# Autodesk Inventor assembly: アーム3
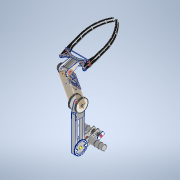
[picture p0: Inventor's stored thumbnail of the model, 180x180]
Saved by Autodesk Inventor 2021 (Build 250183000, 183)
## iProperties
Created: 2022-02-03
Part Number: アーム3
Document SubType Name: Assembly
Designer: hirohumi
Mass: 1757.85 g
Surface Area: 6806.39 cm^2
Volume: 1186.66 cm^3
Density: 1.48134 g/cm^3
Author: hirohumi
## Documents named in this file (25)
- C:\Users\hirohumi\OneDrive\ドキュメント\ロボ研\2022NHKロボコン\R2_version1\3軸アームver3\アーム3.iam
- C:\Users\hirohumi\OneDrive\ドキュメント\ロボ研\2022NHKロボコン\R2_version1\3軸アームver3\アーム3_角柱1.ipt
- C:\Users\hirohumi\OneDrive\ドキュメント\ロボ研\2022NHKロボコン\R2_version1\3軸アームver3\関節3_側板右.ipt
- C:\Users\hirohumi\OneDrive\ドキュメント\ロボ研\2022NHKロボコン\R2_version1\3軸アームver3\関節3_側板左.ipt
- C:\Users\hirohumi\OneDrive\ドキュメント\ロボ研\2022NHKロボコン\R2_version1\RS-555-71.ipt
- C:\Users\hirohumi\OneDrive\ドキュメント\ロボ研\2022NHKロボコン\R2_version1\3軸アーム\カップリング_軸6mm.ipt
- C:\Users\hirohumi\OneDrive\ドキュメント\ロボ研\2022NHKロボコン\R2_version1\3軸アーム\カップリング_軸8mm_2.5mm.ipt
- C:\Users\hirohumi\OneDrive\ドキュメント\ロボ研\2022NHKロボコン\R2_version1\3軸アーム\軸8-30.ipt
- C:\Users\hirohumi\OneDrive\ドキュメント\ロボ研\2022NHKロボコン\R2_version1\3軸アーム\プーリ_歯数15.ipt
- C:\Users\hirohumi\OneDrive\ドキュメント\ロボ研\2022NHKロボコン\R2_version1\3軸アーム\プーリ_歯数15_2.5mm.ipt
- C:\Users\hirohumi\OneDrive\ドキュメント\ロボ研\2022NHKロボコン\R2_version1\3軸アーム\カップリング_軸8mm.ipt
- C:\Users\hirohumi\OneDrive\ドキュメント\ロボ研\2022NHKロボコン\R2_version1\3軸アーム\AMT102Normal\CUI_DEVICES_AMT102-0048-N8000-S.iam
- C:\Users\hirohumi\OneDrive\ドキュメント\ロボ研\2022NHKロボコン\R2_version1\3軸アーム\エンコーダマウント.ipt
- C:\Users\hirohumi\OneDrive\ドキュメント\ロボ研\2022NHKロボコン\R2_version1\3軸アームver2\関節3_プーリ側板.ipt
- C:\Users\hirohumi\OneDrive\ドキュメント\ロボ研\2022NHKロボコン\R2_version1\3軸アーム\ベアリングフランジ付き.ipt
- C:\Users\hirohumi\OneDrive\ドキュメント\ロボ研\2022NHKロボコン\R2_version1\3軸アーム\ギア_歯数50.ipt
- C:\Users\hirohumi\OneDrive\ドキュメント\ロボ研\2022NHKロボコン\R2_version1\RS-775GM104 v1.ipt
- C:\Users\hirohumi\OneDrive\ドキュメント\ロボ研\2022NHKロボコン\R2_version1\3軸アームver3\関節3_前側板.ipt
- C:\Users\hirohumi\OneDrive\ドキュメント\ロボ研\2022NHKロボコン\R2_version1\3軸アーム\プーリ_歯数60.ipt
- C:\Users\hirohumi\OneDrive\ドキュメント\ロボ研\2022NHKロボコン\R2_version1\3軸アーム\関節1_プーリ2個.iam
- C:\Users\hirohumi\OneDrive\ドキュメント\ロボ研\2022NHKロボコン\R2_version1\3軸アーム\軸8-80.ipt
- C:\Users\hirohumi\OneDrive\ドキュメント\ロボ研\2022NHKロボコン\R2_version1\3軸アームver2\関節2_側板.ipt
- C:\Users\hirohumi\OneDrive\ドキュメント\ロボ研\2022NHKロボコン\R2_version1\3軸アームver2\関節2_上板.ipt
- C:\Users\hirohumi\OneDrive\ドキュメント\ロボ研\2022NHKロボコン\R2_version1\R2_ハンド.iam
- C:\Users\hirohumi\OneDrive\ドキュメント\ロボ研\2022NHKロボコン\R2_version1\3軸アームver3\軸_6-30.ipt
## Components (50 placed, 24 different names)
1. アーム3_角柱1:1 — 挿入:62, 挿入:63, 挿入:64, 挿入:65, 挿入:81, 挿入:83, 挿入:85
2. アーム3_角柱1:2 — 挿入:82, 挿入:84, 挿入:86
3. 関節3_側板右:1 — 挿入:83, 挿入:84, 挿入:85, 挿入:86, 挿入:87, 挿入:88, 挿入:89, 挿入:90, 挿入:105, 挿入:106, 挿入:109, 挿入:110
4. 関節3_側板左:1 — 挿入:81, 挿入:82, 挿入:95, 挿入:96, 挿入:97, 挿入:98, 挿入:99, 挿入:100
5. RS-555-71:1 — 挿入:100
6. カップリング_軸6mm:1
7. カップリング_軸8mm_2.5mm:1
8. 軸8-30:1
9. プーリ_歯数15:1
10. プーリ_歯数15_2.5mm:1
11. カップリング_軸8mm:1 — 挿入:108
12. CUI_DEVICES_AMT102-0048-N8000-S:1 [sub-assembly]
13. エンコーダマウント:1 — 挿入:98, 挿入:99
14. 関節3_プーリ側板:1 — 挿入:91, 挿入:92, 挿入:93, 挿入:94
15. ベアリングフランジ付き:1 — 挿入:107
16. ギア_歯数50:1 — 挿入:109, 挿入:110
17. RS-775GM104 v1:1 — 挿入:89, 挿入:90
18. カップリング_軸8mm:2
19. カップリング_軸8mm_2.5mm:2
20. プーリ_歯数15:2
21. プーリ_歯数15_2.5mm:2 — 挿入:107
22. カップリング_軸8mm:3
23. CUI_DEVICES_AMT102-0048-N8000-S:2 [sub-assembly]
24. エンコーダマウント:2 — 挿入:87, 挿入:88
25. ベアリングフランジ付き:2 — 挿入:97
26. 関節3_プーリ側板:2 — 挿入:101, 挿入:102, 挿入:103, 挿入:104
27. ベアリングフランジ付き:3 — 挿入:108
28. 関節3_前側板:1 — 挿入:64, 挿入:65, 挿入:67
29. 関節3_前側板:2 — 挿入:62, 挿入:63, 挿入:66
30. ベアリングフランジ付き:4 — 挿入:66, メイト:3, メイト:6
31. ベアリングフランジ付き:5 — 挿入:67
32. プーリ_歯数60:1 — メイト:6
33. プーリ_歯数60:2 — 挿入:76, 挿入:77
34. 関節1_プーリ2個:1 [sub-assembly] — 挿入:78
35. 軸8-80:1
36. 軸8-80:2
37. 関節2_側板:1 — 挿入:74, 挿入:75, 挿入:76, 挿入:77, 挿入:79, メイト:5
38. 関節2_側板:2 — 挿入:80
39. 軸8-80:3 — 挿入:75, メイト:4
40. 軸8-80:4 — 挿入:74, メイト:3, 挿入:78
41. 関節2_上板:1 — 挿入:79, 挿入:80
42. R2_ハンド:1 [sub-assembly] — メイト:4, メイト:5
43. 軸_6-30:1 — 挿入:91, 挿入:95
44. 軸_6-30:2 — 挿入:92
45. 軸_6-30:3 — 挿入:93, 挿入:96
46. 軸_6-30:4 — 挿入:94
47. 軸_6-30:5 — 挿入:104
48. 軸_6-30:6 — 挿入:103
49. 軸_6-30:7 — 挿入:102, 挿入:106
50. 軸_6-30:8 — 挿入:101, 挿入:105
## Relationships (74: Insert 70, Mate 4)
- [Insert]: カップリング_軸6mm:1 ↔ カップリング_軸8mm_2.5mm:1
- [Insert]: カップリング_軸6mm:1 ↔ カップリング_軸8mm_2.5mm:1
- [Insert]: RS-555-71:1 ↔ カップリング_軸6mm:1
- [Insert]: カップリング_軸6mm:1 ↔ 軸8-30:1
- [Insert]: プーリ_歯数15:1 ↔ プーリ_歯数15_2.5mm:1
- [Insert]: プーリ_歯数15:1 ↔ プーリ_歯数15_2.5mm:1
- [Insert]: プーリ_歯数15:1 ↔ カップリング_軸8mm:1
- [Insert]: プーリ_歯数15:1 ↔ カップリング_軸8mm:1
- [Insert]: CUI_DEVICES_AMT102-0048-N8000-S:1 ↔ エンコーダマウント:1
- [Insert]: CUI_DEVICES_AMT102-0048-N8000-S:1 ↔ エンコーダマウント:1
- [Insert]: 関節3_プーリ側板:1 ↔ ベアリングフランジ付き:1
- [Insert]: カップリング_軸8mm:2 ↔ カップリング_軸8mm_2.5mm:2
- [Insert]: カップリング_軸8mm:2 ↔ カップリング_軸8mm_2.5mm:2
- [Insert]: RS-775GM104 v1:1 ↔ カップリング_軸8mm_2.5mm:2
- [Insert]: プーリ_歯数15:2 ↔ プーリ_歯数15_2.5mm:2
- [Insert]: プーリ_歯数15:2 ↔ プーリ_歯数15_2.5mm:2
- [Insert]: プーリ_歯数15:2 ↔ カップリング_軸8mm:3
- [Insert]: プーリ_歯数15:2 ↔ カップリング_軸8mm:3
- [Insert]: CUI_DEVICES_AMT102-0048-N8000-S:2 ↔ エンコーダマウント:2
- [Insert]: CUI_DEVICES_AMT102-0048-N8000-S:2 ↔ エンコーダマウント:2
- [Insert]: 関節3_プーリ側板:2 ↔ ベアリングフランジ付き:3
- 挿入:62 [Insert]: アーム3_角柱1:1 ↔ 関節3_前側板:2
- 挿入:63 [Insert]: アーム3_角柱1:1 ↔ 関節3_前側板:2
- 挿入:64 [Insert]: アーム3_角柱1:1 ↔ 関節3_前側板:1
- 挿入:65 [Insert]: アーム3_角柱1:1 ↔ 関節3_前側板:1
- 挿入:66 [Insert]: 関節3_前側板:2 ↔ ベアリングフランジ付き:4
- 挿入:67 [Insert]: 関節3_前側板:1 ↔ ベアリングフランジ付き:5
- [Insert]: プーリ_歯数60:1 ↔ プーリ_歯数60:2
- [Insert]: プーリ_歯数60:1 ↔ プーリ_歯数60:2
- [Insert]: 軸8-80:1 ↔ 関節2_側板:1
- [Insert]: 軸8-80:2 ↔ 関節2_側板:1
- [Insert]: 軸8-80:1 ↔ 関節2_側板:2
- [Insert]: 軸8-80:2 ↔ 関節2_側板:2
- 挿入:74 [Insert]: 関節2_側板:1 ↔ 軸8-80:4
- 挿入:75 [Insert]: 関節2_側板:1 ↔ 軸8-80:3
- メイト:3 [Mate]: ベアリングフランジ付き:4 ↔ 軸8-80:4
- 挿入:76 [Insert]: プーリ_歯数60:2 ↔ 関節2_側板:1
- 挿入:77 [Insert]: プーリ_歯数60:2 ↔ 関節2_側板:1
- 挿入:78 [Insert]: 関節1_プーリ2個:1 ↔ 軸8-80:4
- 挿入:79 [Insert]: 関節2_側板:1 ↔ 関節2_上板:1
- 挿入:80 [Insert]: 関節2_側板:2 ↔ 関節2_上板:1
- メイト:4 [Mate]: 軸8-80:3 ↔ R2_ハンド:1
- メイト:5 [Mate]: 関節2_側板:1 ↔ R2_ハンド:1
- メイト:6 [Mate]: ベアリングフランジ付き:4 ↔ プーリ_歯数60:1
- 挿入:81 [Insert]: アーム3_角柱1:1 ↔ 関節3_側板左:1
- 挿入:82 [Insert]: アーム3_角柱1:2 ↔ 関節3_側板左:1
- 挿入:83 [Insert]: アーム3_角柱1:1 ↔ 関節3_側板右:1
- 挿入:84 [Insert]: アーム3_角柱1:2 ↔ 関節3_側板右:1
- 挿入:85 [Insert]: アーム3_角柱1:1 ↔ 関節3_側板右:1
- 挿入:86 [Insert]: アーム3_角柱1:2 ↔ 関節3_側板右:1
- 挿入:87 [Insert]: 関節3_側板右:1 ↔ エンコーダマウント:2
- 挿入:88 [Insert]: 関節3_側板右:1 ↔ エンコーダマウント:2
- 挿入:89 [Insert]: 関節3_側板右:1 ↔ RS-775GM104 v1:1
- 挿入:90 [Insert]: 関節3_側板右:1 ↔ RS-775GM104 v1:1
- 挿入:91 [Insert]: 関節3_プーリ側板:1 ↔ 軸_6-30:1
- 挿入:92 [Insert]: 関節3_プーリ側板:1 ↔ 軸_6-30:2
- 挿入:93 [Insert]: 関節3_プーリ側板:1 ↔ 軸_6-30:3
- 挿入:94 [Insert]: 関節3_プーリ側板:1 ↔ 軸_6-30:4
- 挿入:95 [Insert]: 関節3_側板左:1 ↔ 軸_6-30:1
- 挿入:96 [Insert]: 関節3_側板左:1 ↔ 軸_6-30:3
- 挿入:97 [Insert]: 関節3_側板左:1 ↔ ベアリングフランジ付き:2
- 挿入:98 [Insert]: 関節3_側板左:1 ↔ エンコーダマウント:1
- 挿入:99 [Insert]: 関節3_側板左:1 ↔ エンコーダマウント:1
- 挿入:100 [Insert]: 関節3_側板左:1 ↔ RS-555-71:1
- 挿入:101 [Insert]: 関節3_プーリ側板:2 ↔ 軸_6-30:8
- 挿入:102 [Insert]: 関節3_プーリ側板:2 ↔ 軸_6-30:7
- 挿入:103 [Insert]: 関節3_プーリ側板:2 ↔ 軸_6-30:6
- 挿入:104 [Insert]: 関節3_プーリ側板:2 ↔ 軸_6-30:5
- 挿入:105 [Insert]: 関節3_側板右:1 ↔ 軸_6-30:8
- 挿入:106 [Insert]: 関節3_側板右:1 ↔ 軸_6-30:7
- 挿入:107 [Insert]: ベアリングフランジ付き:1 ↔ プーリ_歯数15_2.5mm:2
- 挿入:108 [Insert]: カップリング_軸8mm:1 ↔ ベアリングフランジ付き:3
- 挿入:109 [Insert]: 関節3_側板右:1 ↔ ギア_歯数50:1
- 挿入:110 [Insert]: 関節3_側板右:1 ↔ ギア_歯数50:1
## Named parameters: d62_d47 = 0 mm, d63_d48 = 0 mm, d64_d49 = 0 mm, d65_d51 = 0 mm, d57_d55 = 0 mm, d58_d56 = 0 mm, d59_d53 = 0 mm, d60_d54 = 0 mm, d81_d4 = 0 mm, d86_d5 = 0 mm, d87_d0 = 0 mm, d88_d1 = 0 mm, d89_d2 = 0 mm, d90_d3 = 0 mm
